# Autodesk Inventor assembly: full intake
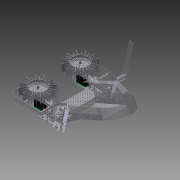
[picture p0: Inventor's stored thumbnail of the model, 180x180]
Saved by Autodesk Inventor 2014 SP1 (Build 180222100, 222)
## iProperties
Created: 2013-10-24
Part Number: full intake
Document SubType Name: Assembly
Designer: RyanHughes
Author: RyanHughes
## Documents named in this file (9)
- C:\Users\Ryan\Desktop\sw\toss up 2ed A bot\intake\full intake.iam
- C:\Users\Ryan\Desktop\sw\lib\Aperture VEX CAD Library\Metal\Plate\5 x 25.ipt
- C:\Users\Ryan\Desktop\sw\toss up 2ed A bot\intake\flip down main.iam
- C:\Users\Ryan\Desktop\sw\toss up 2ed A bot\intake\motor holder.iam
- C:\Users\Ryan\Desktop\sw\toss up 2ed A bot\intake\flappy roller.iam
- C:\Users\Ryan\Desktop\sw\toss up 2ed A bot\intake\flip down main_MIR.iam
- C:\Users\Ryan\Desktop\sw\toss up 2ed A bot\intake\buckies poly\sled.iam
- C:\Users\Ryan\Desktop\sw\toss up 2ed A bot\intake\side guard.iam
- C:\Users\Ryan\Desktop\sw\toss up 2ed A bot\intake\small rail assmb.iam
## Components (12 placed, 8 different names)
1. 5 x 25:1 — Mate:1, Flush:1, Flush:2, Mate:2, Mate:3, Mate:4, Mate:5, Mate:8, Mate:9, Mate:11, Flush:3, Mate:14, Flush:5, Flush:6, Mate:42
2. flip down main:1 [sub-assembly] — Mate:1, Flush:1, Flush:2, Mate:20, Mate:25, Angle:1
3. motor holder:1 [sub-assembly] — Mate:2, Mate:3, Mate:4, Mate:5, Mate:6, Mate:7, Mate:26, Mate:27, Mate:28, Mate:29, Mate:37, Mate:38, Mate:39, Mate:40
4. flappy roller:1 [sub-assembly] — Mate:6, Mate:7
5. motor holder:2 [sub-assembly] — Mate:8, Mate:9, Mate:11, Mate:12, Mate:13, Mate:30, Mate:31, Mate:32, Mate:34, Mate:36, Mate:42
6. flappy roller:2 [sub-assembly] — Mate:12, Mate:13
7. flip down main_MIR:1 [sub-assembly] — Mate:14, Flush:5, Mate:22, Mate:23, Mate:24, Flush:6, Angle:1
8. sled:1 [sub-assembly] — Mate:20, Mate:22, Mate:23, Mate:24, Mate:25
9. side guard:1 [sub-assembly] — Mate:26, Mate:27, Mate:28, Mate:29
10. side guard:2 [sub-assembly] — Mate:30, Mate:31, Mate:32, Mate:33, Mate:35
11. small rail assmb:1 [sub-assembly] — Mate:33, Mate:34, Mate:35, Mate:36
12. small rail assmb:2 [sub-assembly] — Mate:37, Mate:38, Mate:39, Mate:40
## Relationships (40: Mate 34, Flush 5, Angle 1)
- Mate:1: 5 x 25:1 ↔ flip down main:1
- Flush:1: 5 x 25:1 ↔ flip down main:1
- Flush:2: 5 x 25:1 ↔ flip down main:1
- Mate:2: 5 x 25:1 ↔ motor holder:1
- Mate:3 (2.3114 mm): 5 x 25:1 ↔ motor holder:1
- Mate:4 (2.3114 mm): 5 x 25:1 ↔ motor holder:1
- Mate:5 (2.3114 mm): 5 x 25:1 ↔ motor holder:1
- Mate:6: motor holder:1 ↔ flappy roller:1
- Mate:7: motor holder:1 ↔ flappy roller:1
- Mate:8: 5 x 25:1 ↔ motor holder:2
- Mate:9 (2.3114 mm): 5 x 25:1 ↔ motor holder:2
- Mate:11 (2.3114 mm): 5 x 25:1 ↔ motor holder:2
- Mate:12: motor holder:2 ↔ flappy roller:2
- Mate:13: motor holder:2 ↔ flappy roller:2
- Flush:3 (-158.75 mm): 5 x 25:1
- Mate:14: 5 x 25:1 ↔ flip down main_MIR:1
- Flush:5: 5 x 25:1 ↔ flip down main_MIR:1
- Mate:20 (2.3114 mm): flip down main:1 ↔ sled:1
- Mate:22 (2.3114 mm): flip down main_MIR:1 ↔ sled:1
- Mate:23: flip down main_MIR:1 ↔ sled:1
- Mate:24 (2.3114 mm): flip down main_MIR:1 ↔ sled:1
- Mate:25 (2.3114 mm): flip down main:1 ↔ sled:1
- Mate:26: motor holder:1 ↔ side guard:1
- Mate:27 (2.3114 mm): motor holder:1 ↔ side guard:1
- Mate:28 (2.3114 mm): motor holder:1 ↔ side guard:1
- Mate:29: motor holder:1 ↔ side guard:1
- Mate:30: motor holder:2 ↔ side guard:2
- Mate:31: motor holder:2 ↔ side guard:2
- Mate:32 (2.3114 mm): motor holder:2 ↔ side guard:2
- Flush:6: 5 x 25:1 ↔ flip down main_MIR:1
- Angle:1 (0 deg): flip down main:1 ↔ flip down main_MIR:1
- Mate:33: side guard:2 ↔ small rail assmb:1
- Mate:34 (2.3114 mm): motor holder:2 ↔ small rail assmb:1
- Mate:35 (2.3114 mm): side guard:2 ↔ small rail assmb:1
- Mate:36 (2.3114 mm): motor holder:2 ↔ small rail assmb:1
- Mate:37: motor holder:1 ↔ small rail assmb:2
- Mate:38 (2.3114 mm): motor holder:1 ↔ small rail assmb:2
- Mate:39 (2.3114 mm): motor holder:1 ↔ small rail assmb:2
- Mate:40 (2.3114 mm): motor holder:1 ↔ small rail assmb:2
- Mate:42 (2.3114 mm): 5 x 25:1 ↔ motor holder:2
## Named parameters: q = 2.3114 mm
